# Autodesk Inventor assembly: FTC 1
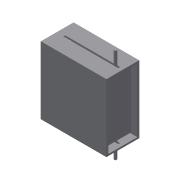
[picture p0: Inventor's stored thumbnail of the model, 180x180]
Saved by Autodesk Inventor 2013 (Build 170138000, 138)
## iProperties
Created: 2013-09-11
Part Number: FTC 1
Document SubType Name: Assembly
Designer: Connor
Author: Connor
## Documents named in this file (3)
- C:\Users\Connor\Desktop\FTC 1.iam
- C:\Users\Connor\Desktop\BOX.ipt
- C:\Users\Connor\Desktop\Pushewr.ipt
## Components (2 placed, 2 different names)
1. BOX:1 — Mate:1
2. Pushewr:1 — Mate:1
## Relationships (1: Mate 1)
- Mate:1 (2.286 mm): BOX:1 ↔ Pushewr:1
